# Autodesk Inventor assembly: box
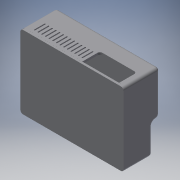
[picture p0: Inventor's stored thumbnail of the model, 180x180]
Saved by Autodesk Inventor 2019 (Build 230136000, 136)
## iProperties
Created: 2021-11-14
Part Number: box
Document SubType Name: Assembly
Designer: Tiarnan Rice
Author: Tiarnan Rice
## Documents named in this file (3)
- C:\Users\Tiarnan Rice.DESKTOP-42BQHLM\Desktop\AirQualityMonitor\enclosure\box.iam
- C:\Users\Tiarnan Rice.DESKTOP-42BQHLM\Desktop\AirQualityMonitor\enclosure\box.ipt
- C:\Users\Tiarnan Rice.DESKTOP-42BQHLM\Desktop\AirQualityMonitor\enclosure\lid.ipt
## Components (2 placed, 2 different names)
1. box:1 — Mate:1, Flush:1, Flush:2
2. lid:1 — Mate:1, Flush:1, Flush:2
## Relationships (3: Flush 2, Mate 1)
- Mate:1: box:1 ↔ lid:1
- Flush:1: box:1 ↔ lid:1
- Flush:2: box:1 ↔ lid:1
